# Autodesk Inventor assembly: assembily_v2
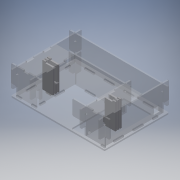
[picture p0: Inventor's stored thumbnail of the model, 180x180]
Saved by Autodesk Inventor 2017.2 (Build 212233000, 233)
## iProperties
Created: 2017-06-09
Part Number: assembily_v2
Document SubType Name: Assembly
Designer: SandeepSH
Author: SandeepSH
## Documents named in this file (14)
- C:\Users\SandeepSH\Dropbox\MSC\Project\inventor\lcv1\assembily_v2.iam
- C:\Users\SandeepSH\Dropbox\MSC\Project\inventor\lcv1\base_v2.ipt
- C:\Users\SandeepSH\Dropbox\MSC\Project\inventor\lcv1\cham_right_v2.ipt
- C:\Users\SandeepSH\Dropbox\MSC\Project\inventor\lcv1\cham_back_v2.ipt
- C:\Users\SandeepSH\Dropbox\MSC\Project\inventor\lcv1\front_right_v2.ipt
- C:\Users\SandeepSH\Dropbox\MSC\Project\inventor\lcv1\cham_left_v2.ipt
- C:\Users\SandeepSH\Dropbox\MSC\Project\inventor\lcv1\front_left_v2.ipt
- C:\Users\SandeepSH\Dropbox\MSC\Project\inventor\lcv1\side_v2.ipt
- C:\Users\SandeepSH\Dropbox\MSC\Project\inventor\lcv1\back_v2.ipt
- C:\Users\SandeepSH\Dropbox\MSC\Project\inventor\lcv1\top_right_v2.ipt
- C:\Users\SandeepSH\Dropbox\MSC\Project\inventor\lcv1\hollow_mount.ipt
- C:\Users\SandeepSH\Dropbox\MSC\Project\inventor\lcv1\fill_mount.ipt
- C:\Users\SandeepSH\Dropbox\MSC\Project\inventor\lcv1\fill_mount _right.ipt
- C:\Users\SandeepSH\Dropbox\MSC\Project\inventor\lcv1\hollow_mount_right.ipt
## Components (17 placed, 13 different names)
1. base_v2:1 — Mate:1, Mate:2, Mate:3, Mate:6, Mate:7, Mate:8, Mate:9, Mate:10, Mate:11, Mate:12, Mate:13, Mate:14, Mate:15, Mate:16, Mate:17, Mate:20, Mate:21, Mate:22, Mate:23, Mate:24, Mate:25
2. front_right_v2:1 — Mate:1, Mate:6
3. cham_back_v2:1 — Mate:2, Mate:3, Mate:4, Mate:5, Mate:7
4. cham_right_v2:1 — Mate:4, Mate:5, Mate:28, Mate:29, Mate:30, Mate:31, Mate:32, Mate:33, Mate:34, Mate:35
5. cham_left_v2:1 — Mate:8, Mate:9
6. front_left_v2:1 — Mate:10, Mate:11, Mate:26, Mate:27
7. side_v2:1 — Mate:12, Mate:13
8. side_v2:2 — Mate:14, Mate:15
9. back_v2:1 — Mate:16, Mate:17
10. hollow_mount:1 — Mate:22, Mate:23
11. fill_mount:1 — Mate:24, Mate:25
12. fill_mount:2 — Mate:20, Mate:21
13. top_right_v2:2 — Mate:26, Mate:27
14. fill_mount _right:1 — Mate:30, Mate:31
15. fill_mount _right:2 — Mate:32, Mate:33
16. hollow_mount_right:1 — Mate:28, Mate:29
17. top_right_v2:3 — Mate:34, Mate:35
## Relationships (33: Mate 33)
- Mate:1: base_v2:1 ↔ front_right_v2:1
- Mate:2: base_v2:1 ↔ cham_back_v2:1
- Mate:3: base_v2:1 ↔ cham_back_v2:1
- Mate:4: cham_back_v2:1 ↔ cham_right_v2:1
- Mate:5: cham_back_v2:1 ↔ cham_right_v2:1
- Mate:6: base_v2:1 ↔ front_right_v2:1
- Mate:7: base_v2:1 ↔ cham_back_v2:1
- Mate:8: base_v2:1 ↔ cham_left_v2:1
- Mate:9: base_v2:1 ↔ cham_left_v2:1
- Mate:10: base_v2:1 ↔ front_left_v2:1
- Mate:11: base_v2:1 ↔ front_left_v2:1
- Mate:12: base_v2:1 ↔ side_v2:1
- Mate:13: base_v2:1 ↔ side_v2:1
- Mate:14: base_v2:1 ↔ side_v2:2
- Mate:15: base_v2:1 ↔ side_v2:2
- Mate:16: base_v2:1 ↔ back_v2:1
- Mate:17: base_v2:1 ↔ back_v2:1
- Mate:20: base_v2:1 ↔ fill_mount:2
- Mate:21: base_v2:1 ↔ fill_mount:2
- Mate:22: base_v2:1 ↔ hollow_mount:1
- Mate:23: base_v2:1 ↔ hollow_mount:1
- Mate:24: base_v2:1 ↔ fill_mount:1
- Mate:25: base_v2:1 ↔ fill_mount:1
- Mate:26: front_left_v2:1 ↔ top_right_v2:2
- Mate:27: front_left_v2:1 ↔ top_right_v2:2
- Mate:28: cham_right_v2:1 ↔ hollow_mount_right:1
- Mate:29: cham_right_v2:1 ↔ hollow_mount_right:1
- Mate:30: cham_right_v2:1 ↔ fill_mount _right:1
- Mate:31: cham_right_v2:1 ↔ fill_mount _right:1
- Mate:32: cham_right_v2:1 ↔ fill_mount _right:2
- Mate:33: cham_right_v2:1 ↔ fill_mount _right:2
- Mate:34: cham_right_v2:1 ↔ top_right_v2:3
- Mate:35: cham_right_v2:1 ↔ top_right_v2:3
